# Autodesk Inventor assembly: TornilloKK8610P540A1F000_FILE_1
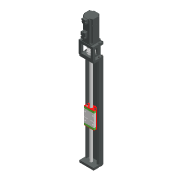
[picture p0: Inventor's stored thumbnail of the model, 180x180]
Saved by Autodesk Inventor 2021 (Build 250183000, 183)
## iProperties
Company: CADClick - www.CADClick.com
Created: 2021-08-22
Part Number: TornilloKK8610P540A1F000_FILE_1
Description: STEP AP214
Document SubType Name: Assembly
Designer: Santiago Suárez
Authority: unknown authorization
Title: cctmp_A6BB2A8F-F6D2-46C5-9C22-2770F8FE21AB_2021_08_22_08_09_33_0365..stp
Author: HIWIN GmbH
Revision Number: NONE
Preprocessor: Spatial InterOp 3D
## Documents named in this file (5)
- C:\Users\Santiago Suárez\Documents\GitHub\Dis.-Mecatronico-E6\inventor proyecto\Guias\TornilloKK8610P540A1F000_FILE_1.iam
- C:\Users\Santiago Suárez\Documents\GitHub\Dis.-Mecatronico-E6\inventor proyecto\Guias\TornilloKK8610P540A1F000_FILE_1.ipt
- C:\Users\Santiago Suárez\Documents\GitHub\Dis.-Mecatronico-E6\inventor proyecto\Guias\TornilloKK8610P540A1F000_FILE.ipt
- C:\Users\Santiago Suárez\Documents\GitHub\Dis.-Mecatronico-E6\inventor proyecto\Guias\MotorFRLS202B606A_FILE_2.ipt
- C:\Users\Santiago Suárez\Documents\GitHub\Dis.-Mecatronico-E6\inventor proyecto\Guias\gsf_gr__2_d8_b___d14_b.ipt
## Components (4 placed, 4 different names)
1. TornilloKK8610P540A1F000_FILE_1 — Slider:1
2. TornilloKK8610P540A1F000_FILE — Slider:1
3. MotorFRLS202B606A_FILE_2:1 — Rotational:1
4. gsf_gr__2_d8_b___d14_b:1 — Rotational:1
## Relationships (2: TranslationJoint 1, RevoluteJoint 1)
- Slider:1 [TranslationJoint] (6 mm): TornilloKK8610P540A1F000_FILE_1 ↔ TornilloKK8610P540A1F000_FILE
- Rotational:1 [RevoluteJoint]: MotorFRLS202B606A_FILE_2:1 ↔ gsf_gr__2_d8_b___d14_b:1
